# Autodesk Inventor assembly: 1x10
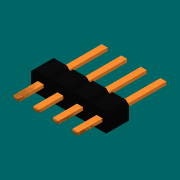
[picture p0: Inventor's stored thumbnail of the model, 180x180]
Saved by Autodesk Inventor 2016 (Build 200138000, 138)
## iProperties
Created: 2014-07-19
Part Number: 1x10
Document SubType Name: Assembly
Designer: Sawaiz Syed
Author: Sawaiz Syed
## Documents named in this file (2)
- C:\Users\sawaiz\oneDrive\projects\splitFlapDisplay\electronics\cad\component\1x4.iam
- C:\Users\sawaiz\oneDrive\projects\splitFlapDisplay\electronics\cad\component\1x1.iam
## Components (4 placed, 1 different names)
1. 1x1:1 [sub-assembly]
2. 1x1:2 [sub-assembly]
3. 1x1:3 [sub-assembly]
4. 1x1:4 [sub-assembly]
## Component patterns: (4 elements, first: 1x1:1)
